# Autodesk Inventor assembly: Y Axis
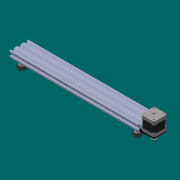
[picture p0: Inventor's stored thumbnail of the model, 180x180]
Saved by Autodesk Inventor 2016 (Build 200138000, 138)
## iProperties
Created: 2015-06-04
Part Number: Y Axis
Document SubType Name: Assembly
Designer: Sawaiz Syed
Author: Sawaiz Syed
## Documents named in this file (4)
- C:\Users\Sawaiz\Documents\data\projects\cncBlackBox\yAxis\yAxis.iam
- C:\Users\Sawaiz\Documents\data\projects\cncBlackBox\yAxis\slider\slider.iam
- C:\Users\Sawaiz\Documents\data\projects\cncBlackBox\yAxis\slider\motorizedSlider.iam
- C:\Users\Sawaiz\Documents\data\projects\cncBlackBox\yAxis\yAxisVSlot.ipt
## Components (3 placed, 3 different names)
1. motorizedSlider:1 [sub-assembly] — Flush:1, Mate:3, Flush:4
2. slider:1 [sub-assembly] — Flush:1, Mate:1, Flush:3, Flush:4, Mate:4
3. yAxisVSlot:1 — Mate:1, Mate:3, Flush:3, Mate:4
## Relationships (6: Flush 3, Mate 3)
- Flush:1: motorizedSlider:1 ↔ slider:1
- Mate:1: slider:1 ↔ yAxisVSlot:1
- Mate:3: motorizedSlider:1 ↔ yAxisVSlot:1
- Flush:3 (17.8 mm): slider:1 ↔ yAxisVSlot:1
- Flush:4: motorizedSlider:1 ↔ slider:1
- Mate:4 (0.5 mm): slider:1 ↔ yAxisVSlot:1
